# Autodesk Inventor assembly: CLB_059_ScissorLiftBottomBrackets
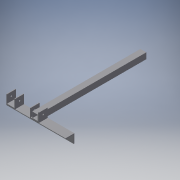
[picture p0: Inventor's stored thumbnail of the model, 180x180]
Saved by Autodesk Inventor 2018.3 (Build 223284000, 284)
## iProperties
Created: 2020-02-17
Part Number: CLB_059_ScissorLiftBottomBrackets
Document SubType Name: Assembly
Designer: 22perngrac
Author: 22perngrac
## Documents named in this file (4)
- C:\Users\22perngrac\Documents\GrabCAD\Infinite Recharge 2020\Build season\CLB_063_ScissorLiftFixedEndBrackets.iam
- C:\Users\22perngrac\Documents\GrabCAD\Infinite Recharge 2020\Build season\CLB_062_OutsideLBracket.ipt
- C:\Users\22perngrac\Documents\GrabCAD\Infinite Recharge 2020\Build season\CLB_064_ScissorLiftUBracket.ipt
- C:\Users\22perngrac\Documents\GrabCAD\Infinite Recharge 2020\Build season\CLB_075_ScissorBase.ipt
## Components (4 placed, 3 different names)
1. CLB_062_OutsideLBracket:1 — Mate:12, Flush:1, Flush:4, Mate:14, Mate:15, Mate:19
2. CLB_064_ScissorLiftUBracket:2 — Mate:12, Flush:1, Flush:4, Flush:5, Flush:6
3. CLB_075_ScissorBase:1 — Mate:20, Flush:7, Mate:21
4. CLB_064_ScissorLiftUBracket:3 — Mate:19, Flush:5, Flush:6, Mate:20, Flush:7, Mate:21
## Relationships (11: Mate 6, Flush 5)
- Mate:12: CLB_062_OutsideLBracket:1 ↔ CLB_064_ScissorLiftUBracket:2
- Flush:1: CLB_062_OutsideLBracket:1 ↔ CLB_064_ScissorLiftUBracket:2
- Flush:4: CLB_062_OutsideLBracket:1 ↔ CLB_064_ScissorLiftUBracket:2
- Mate:14: CLB_062_OutsideLBracket:1
- Mate:15: CLB_062_OutsideLBracket:1
- Mate:19: CLB_062_OutsideLBracket:1 ↔ CLB_064_ScissorLiftUBracket:3
- Flush:5: CLB_064_ScissorLiftUBracket:2 ↔ CLB_064_ScissorLiftUBracket:3
- Flush:6 (101.6 mm): CLB_064_ScissorLiftUBracket:2 ↔ CLB_064_ScissorLiftUBracket:3
- Mate:20: CLB_075_ScissorBase:1 ↔ CLB_064_ScissorLiftUBracket:3
- Flush:7: CLB_075_ScissorBase:1 ↔ CLB_064_ScissorLiftUBracket:3
- Mate:21: CLB_075_ScissorBase:1 ↔ CLB_064_ScissorLiftUBracket:3
